# Autodesk Inventor assembly: SSCSM12-8
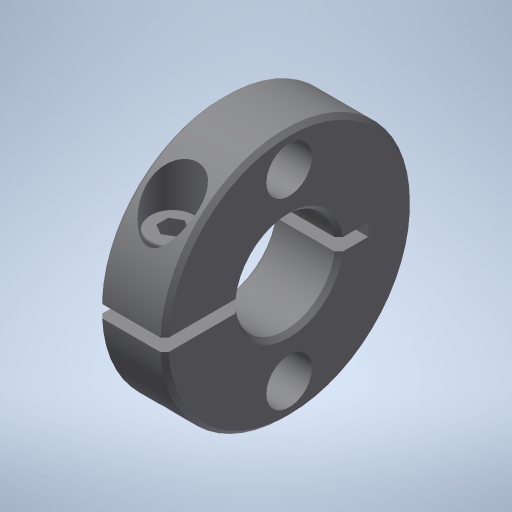
[picture p0: Inventor's stored thumbnail of the model, 512x512]
Saved by Autodesk Inventor 2023.2 (Build 272271030, 271C)
## iProperties
Created: 2023-04-27
Part Number: SSCSM12-8
Catalog Web Link: www.cadenas.de
Description: SCSM, PSCSM, SSCSM, SCSMA, SCSMAW-Set Collars - Slit 2 Hole/2 Tap - Standard Type - 2 Hole Type
Vendor: MISUMI
Document SubType Name: Assembly
Designer: psAdmin
Manufacturer: MISUMI
Mass: 4.07496 g
Surface Area: 29.0447 cm^2
Volume: 4.07496 cm^3
Density: 1 g/cm^3
Category: PARTsolutions
Company: MISUMI
PSOL_IDENT_0: {$CADENAS_DATA/23d-libs/misumi/metric/03_set_collars/scsm_asmtab.prj},210 {VTYP=3D},{STYP=ASSTAB},{N
PSOL_IDENT_1: B=SSCSM12-8},{LINA=SSCSM12-8},{NN=SCSM, PSCSM, SSCSM, SCSMA, SCSMAW},{DATE=30.11.2021 05:42:00},{GEO
PSOL_IDENT_2: MDATE=15.09.2021 05:26:16},{VERSION=},{LINEID=70},{WBVAR=MAT,ST,BS},{WBNUMERIC=BS}  {NB=SSCSM12-8},{
PSOL_IDENT_3: LINA=SSCSM12-8},{KT=DUMMY},{PN=SSCSM12-8},{TYPE=SSCSM},{MAT=304},{ST=-},{ST0='-','-'},{AC=Hexagon So
PSOL_IDENT_4: cket Head Set Screw 1 Pc. (304 Stainless Steel) },{D=12},{BS=8},{B1=8,10,12,15},{D1=30},{M=M3},{THMD=
PSOL_IDENT_5: 3},{THDMIN=2.459},{DD=3.4},{R=3.00},{W=1.5},{X=10.0},{Y=5},{Z=9~10},{S=5.5},{P=22},{C=0.5},{L=12},{M
PSOL_IDENT_6: 1=-},{ZZ=9.5},{PPATH=scsm_templ.prj},{MATA='1045','S45C Equivalent','304','SUS304 Equivalent','2017'
PSOL_IDENT_7: ,'2017 Aluminum Alloy'}
NB: SSCSM12-8
NN: SCSM, PSCSM, SSCSM, SCSMA, SCSMAW
NT: Set Collars - Slit 2 Hole/2 Tap - Standard Type - 2 Hole Type
NBSYN: $PN.
LINA: SSCSM12-8
CATALOG: Misumi
PN: SSCSM12-8
MAT: SUS304 Equivalent
ST: -
AC: Hexagon Socket Head Set Screw 1 Pc. (304 Stainless Steel)
D: 12
BS: 8
D1: 30
M: M3
DD: 3.4
R: 3
W: 1.5
X: 10
Y: 5
Z: 9~10
S: 5.5
P: 22
SUPPLIER: MISUMI
ARTICLENO: SSCSM12-8
BOMINFO: SSCSM12-8
CREATOR: CADENAS GmbH
Title: SSCSM12-8
Author: Cadenas PARTsolutions
Comments: Set Collars - Slit 2 Hole/2 Tap - Standard Type - 2 Hole Type
## Documents named in this file (3)
- C:\Users\haruy\Documents\ロボコン\1年\ER_secondvideo_0314 ver2\ER_0314\SSCSM12-8_Autodesk_Inventor_2022_20230427\AIS2022\SSCSM12-8.iam
- C:\Users\haruy\Documents\ロボコン\1年\ER_secondvideo_0314 ver2\ER_0314\SSCSM12-8_Autodesk_Inventor_2022_20230427\AIS2022\SSCSM12-8b.ipt
- C:\Users\haruy\Documents\ロボコン\1年\ER_secondvideo_0314 ver2\ER_0314\SSCSM12-8_Autodesk_Inventor_2022_20230427\AIS2022\Slotted head cap screw ISO 4762 - M3x12.ipt
## Components (2 placed, 2 different names)
1. SSCSM12-8b:1 — body_screw_Z@1 <-> IP1_Z@2
2. Slotted head cap screw ISO 4762 - M3x12:1 — body_screw_Z@1 <-> IP1_Z@2
## Relationships (1: Mate 1)
- body_screw_Z@1 <-> IP1_Z@2 [Mate]: SSCSM12-8b:1 ↔ Slotted head cap screw ISO 4762 - M3x12:1
